# Autodesk Inventor assembly: KP08
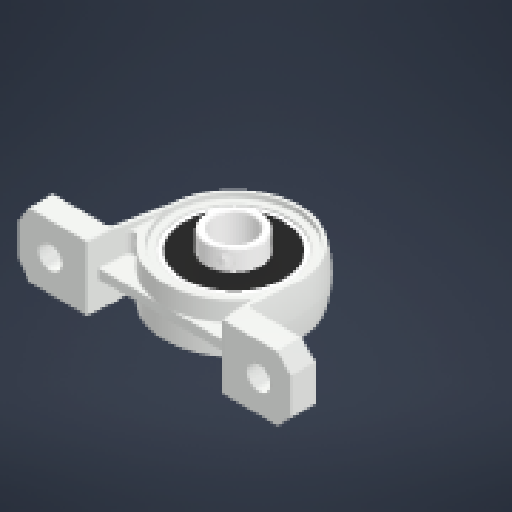
[picture p0: Inventor's stored thumbnail of the model, 512x512]
Saved by Autodesk Inventor 2024 (Build 280153000, 153)
## iProperties
Created: 2017-02-04
Part Number: KP08
Description: STEP AP214
Document SubType Name: Assembly
Designer: user
Sending System: SolidWorks 2016
Preprocessor: SwSTEP 2.0
Title: KP08.STEP
Author: DronnnTM
Revision Number: ANY
## Documents named in this file (3)
- D:\Docs\Robot\3d_v2\default_components\KP08.iam
- D:\Docs\Robot\3d_v2\default_components\KP08\KP08\KP08.ipt
- D:\Docs\Robot\3d_v2\default_components\KP08\KP08\608RS.ipt
## Components (2 placed, 2 different names)
1. KP08_1 — Вставка:1
2. 608RS_2 — Вставка:1
## Relationships (1: Insert 1)
- Вставка:1 [Insert]: KP08_1 ↔ 608RS_2
